# Autodesk Inventor assembly: Control Cylinder
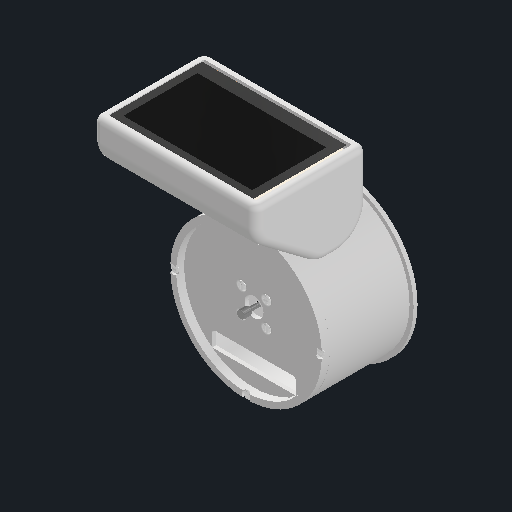
[picture p0: Inventor's stored thumbnail of the model, 512x512]
Saved by Autodesk Inventor 2023 (Build 270158000, 158)
## iProperties
Created: 2023-04-06
Part Number: Control Cylinder
Document SubType Name: Assembly
Designer: vatdu
Author: vatdu
## Documents named in this file (10)
- C:\Users\vatdu\Desktop\CRYSTAL MARK II\Controller Housing\Control Cylinder.iam
- C:\Users\vatdu\Desktop\CRYSTAL MARK II\Controller Housing\Components Base.ipt
- C:\Users\vatdu\Desktop\CRYSTAL MARK II\Controller Housing\Outer Shell.ipt
- C:\Users\vatdu\Desktop\CRYSTAL MARK II\Controller Housing\Motor Holder.ipt
- C:\Users\vatdu\Desktop\CRYSTAL MARK II\Components\Stepper Motor.ipt
- C:\Users\vatdu\Desktop\CRYSTAL MARK II\Components\Raspberry Pi 4\Raspberry Pi 4 Model B.iam
- C:\Users\vatdu\Desktop\CRYSTAL MARK II\Components\Arduino Nano\arduino nano.iam
- C:\Users\vatdu\Desktop\CRYSTAL MARK II\Components\Screw Big.ipt
- C:\Users\vatdu\Desktop\CRYSTAL MARK II\Controller Housing\Screen Mount.ipt
- C:\Users\vatdu\Desktop\CRYSTAL MARK II\Components\Raspberry Pi Screen\Screen.ipt
## Components (20 placed, 9 different names)
1. Components Base:1 — Rotational:1, Rotational:2, Rotational:4, Rotational:8, Rotational:9, Rotational:10, Rotational:11
2. Outer Shell:1 — Rotational:1, Rotational:2, Rotational:4, Rotational:12
3. Stepper Motor:1
4. Raspberry Pi 4 Model B:1 [sub-assembly]
5. arduino nano:1 [sub-assembly]
6. Screw Big:1 — Rotational:8
7. Screw Big:2 — Rotational:9
8. Screw Big:3 — Rotational:10
9. Screw Big:4 — Rotational:11
10. Screw Big:5
11. Screw Big:6
12. Screw Big:7
13. Screw Big:8
14. Screw Big:9
15. Screw Big:10
16. Screw Big:11
17. Screw Big:12
18. Screen:1
19. Motor Holder:1 — Rotational:12, Rotational:13
20. Screen Mount:1 — Rotational:13
## Relationships (9: RevoluteJoint 9)
- Rotational:1 [RevoluteJoint]: Components Base:1 ↔ Outer Shell:1
- Rotational:2 [RevoluteJoint]: Components Base:1 ↔ Outer Shell:1
- Rotational:4 [RevoluteJoint]: Components Base:1 ↔ Outer Shell:1
- Rotational:8 [RevoluteJoint]: Components Base:1 ↔ Screw Big:1
- Rotational:9 [RevoluteJoint]: Components Base:1 ↔ Screw Big:2
- Rotational:10 [RevoluteJoint]: Components Base:1 ↔ Screw Big:3
- Rotational:11 [RevoluteJoint]: Components Base:1 ↔ Screw Big:4
- Rotational:12 [RevoluteJoint]: Outer Shell:1 ↔ Motor Holder:1
- Rotational:13 [RevoluteJoint]: Motor Holder:1 ↔ Screen Mount:1
